# Autodesk Inventor assembly: Y_GANTRY
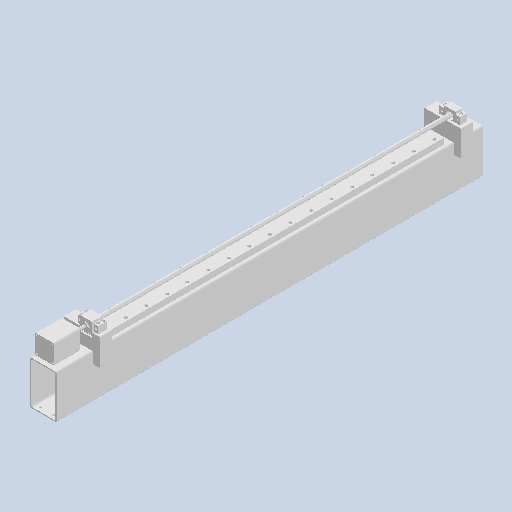
[picture p0: Inventor's stored thumbnail of the model, 512x512]
Saved by Autodesk Inventor 2023 (Build 270158000, 158)
## iProperties
Created: 2022-05-07
Part Number: Y_GANTRY
Document SubType Name: Assembly
Designer: plebbb
Author: plebbb
## Documents named in this file (9)
- D:\Users\plebbb\Desktop\CNC_Project\Y_GANTRY.iam
- D:\Users\plebbb\Desktop\CNC_Project\5x3_Tube.ipt
- D:\Users\plebbb\Desktop\CNC_Project\HGW20CC_Rail_800mm.ipt
- D:\Users\plebbb\Desktop\CNC_Project\BF10.ipt
- D:\Users\plebbb\Desktop\CNC_Project\BK10.ipt
- D:\Users\plebbb\Desktop\CNC_Project\SFU1204-500.ipt
- D:\Users\plebbb\Desktop\CNC_Project\BF10_Spacer.ipt
- D:\Users\plebbb\Desktop\CNC_Project\BK10_Spacer.ipt
- D:\Users\plebbb\Desktop\CNC_Project\Nema23.ipt
## Components (9 placed, 8 different names)
1. 5x3_Tube:1
2. HGW20CC_Rail_800mm:1
3. BF10:1
4. BK10:1
5. SFU1204-500:1
6. BF10_Spacer:1
7. BK10_Spacer:1
8. HGW20CC_Rail_800mm:2
9. Nema23:1
## Relationships (23: Mate 18, Flush 5)
- [Mate]: 5x3_Tube:1 ↔ HGW20CC_Rail_800mm:1
- [Mate]: BK10:1 ↔ SFU1204-500:1
- [Mate]: BK10:1 ↔ SFU1204-500:1
- [Mate]: BF10:1 ↔ SFU1204-500:1
- [Mate]: BF10:1 ↔ SFU1204-500:1
- [Flush] (-10 mm): 5x3_Tube:1 ↔ HGW20CC_Rail_800mm:1
- [Mate]: BK10:1 ↔ BK10_Spacer:1
- [Mate]: BK10:1 ↔ BK10_Spacer:1
- [Mate]: BK10:1 ↔ BK10_Spacer:1
- [Mate]: 5x3_Tube:1 ↔ BK10_Spacer:1
- [Mate]: BF10:1 ↔ BF10_Spacer:1
- [Mate]: BF10:1 ↔ BF10_Spacer:1
- [Mate]: BF10:1 ↔ BF10_Spacer:1
- [Mate]: 5x3_Tube:1 ↔ BF10_Spacer:1
- [Mate]: 5x3_Tube:1 ↔ BF10_Spacer:1
- [Flush] (50 mm): 5x3_Tube:1 ↔ BF10_Spacer:1
- [Mate]: HGW20CC_Rail_800mm:1 ↔ BK10_Spacer:1
- [Mate]: SFU1204-500:1 ↔ Nema23:1
- [Mate]: SFU1204-500:1 ↔ Nema23:1
- [Mate]: 5x3_Tube:1 ↔ HGW20CC_Rail_800mm:2
- [Flush]: HGW20CC_Rail_800mm:1 ↔ HGW20CC_Rail_800mm:2
- [Flush] (28.1 mm): 5x3_Tube:1 ↔ HGW20CC_Rail_800mm:2
- [Flush]: HGW20CC_Rail_800mm:1 ↔ HGW20CC_Rail_800mm:2
